# Autodesk Inventor assembly: Calorímetro
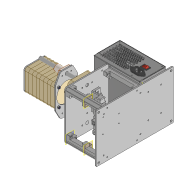
[picture p0: Inventor's stored thumbnail of the model, 180x180]
Saved by Autodesk Inventor 2020 (Build 240168000, 168)
## iProperties
Created: 2022-07-16
Part Number: Calorímetro
Document SubType Name: Assembly
Designer: gabri
Author: gabri
## Documents named in this file (11)
- C:\Users\gabri\OneDrive\Área de Trabalho\Calorimetro 2022\Inventor\Calorímetro.iam
- C:\Users\gabri\OneDrive\Área de Trabalho\Calorimetro 2022\Inventor\Fonte\ATX Power Supply v1.iam
- C:\Users\gabri\OneDrive\Área de Trabalho\Calorimetro 2022\Inventor\Base.ipt
- C:\Users\gabri\OneDrive\Área de Trabalho\Calorimetro 2022\Inventor\parte_superior.iam
- C:\Users\gabri\OneDrive\Área de Trabalho\Calorimetro 2022\Inventor\Montagem_suporte_termopar.iam
- C:\Users\gabri\OneDrive\Área de Trabalho\Calorimetro 2022\Inventor\Peça4.ipt
- C:\Users\gabri\OneDrive\Área de Trabalho\Calorimetro 2022\Inventor\suporte-fonte.ipt
- C:\Users\gabri\OneDrive\Área de Trabalho\Calorimetro 2022\Inventor\suporte_fechamento.ipt
- C:\Users\gabri\OneDrive\Área de Trabalho\Calorimetro 2022\Inventor\suporte_fechamento2.ipt
- C:\Users\gabri\OneDrive\Área de Trabalho\Calorimetro 2022\Inventor\fechamentocima.ipt
- C:\Users\gabri\OneDrive\Área de Trabalho\Calorimetro 2022\Inventor\Mega.ipt
## Components (12 placed, 10 different names)
1. ATX Power Supply v1:1 [sub-assembly] — Coincidência:1, Alinhamento:1, Coincidência:2, Coincidência:5, Coincidência:6, Alinhamento:4, Alinhamento:5, Alinhamento:6, Alinhamento:7
2. Base:1 — Coincidência:7, Alinhamento:6, Alinhamento:7, Coincidência:8, Coincidência:9, Alinhamento:8, Alinhamento:9, Alinhamento:10, Alinhamento:12, Coincidência:10, Coincidência:12, Coincidência:16, Alinhamento:19, Alinhamento:20
3. parte_superior:1 [sub-assembly] — Coincidência:4, Alinhamento:2, Coincidência:13, Alinhamento:17, Alinhamento:18, Coincidência:14
4. Montagem_suporte_termopar:1 [sub-assembly] — Coincidência:4, Coincidência:14, Coincidência:15, Ângulo:1
5. Peça4:1 — Alinhamento:2
6. suporte-fonte:1 — Coincidência:5, Coincidência:6, Coincidência:7, Alinhamento:4, Alinhamento:5, Coincidência:11
7. suporte_fechamento:1 — Coincidência:8, Alinhamento:8, Alinhamento:11, Alinhamento:15
8. suporte_fechamento:2 — Coincidência:9, Alinhamento:9, Alinhamento:10, Alinhamento:11, Alinhamento:13, Alinhamento:16
9. suporte_fechamento2:2 — Alinhamento:12, Coincidência:10, Coincidência:11, Alinhamento:14
10. suporte_fechamento2:3 — Coincidência:12, Alinhamento:13, Alinhamento:14
11. fechamentocima:1 — Alinhamento:15, Alinhamento:16, Coincidência:13, Alinhamento:17, Alinhamento:18, Coincidência:15, Ângulo:1
12. Mega:1 — Coincidência:16, Alinhamento:19, Alinhamento:20
## Relationships (35: Flush 19, Mate 15, Angle 1)
- Coincidência:1 [Mate] (-71 mm): ATX Power Supply v1:1
- Alinhamento:1 [Flush]: ATX Power Supply v1:1
- Coincidência:2 [Mate]: ATX Power Supply v1:1
- Coincidência:4 [Mate]: parte_superior:1 ↔ Montagem_suporte_termopar:1
- Alinhamento:2 [Flush]: parte_superior:1 ↔ Peça4:1
- Coincidência:5 [Mate]: ATX Power Supply v1:1 ↔ suporte-fonte:1
- Coincidência:6 [Mate]: ATX Power Supply v1:1 ↔ suporte-fonte:1
- Coincidência:7 [Mate]: Base:1 ↔ suporte-fonte:1
- Alinhamento:4 [Flush]: ATX Power Supply v1:1 ↔ suporte-fonte:1
- Alinhamento:5 [Flush] (-8 mm): ATX Power Supply v1:1 ↔ suporte-fonte:1
- Alinhamento:6 [Flush] (-13 mm): ATX Power Supply v1:1 ↔ Base:1
- Alinhamento:7 [Flush]: ATX Power Supply v1:1 ↔ Base:1
- Coincidência:8 [Mate]: Base:1 ↔ suporte_fechamento:1
- Coincidência:9 [Mate]: Base:1 ↔ suporte_fechamento:2
- Alinhamento:8 [Flush]: Base:1 ↔ suporte_fechamento:1
- Alinhamento:9 [Flush]: Base:1 ↔ suporte_fechamento:2
- Alinhamento:10 [Flush] (15 mm): Base:1 ↔ suporte_fechamento:2
- Alinhamento:11 [Flush]: suporte_fechamento:1 ↔ suporte_fechamento:2
- Alinhamento:12 [Flush]: Base:1 ↔ suporte_fechamento2:2
- Coincidência:10 [Mate]: Base:1 ↔ suporte_fechamento2:2
- Coincidência:11 [Mate]: suporte-fonte:1 ↔ suporte_fechamento2:2
- Coincidência:12 [Mate]: Base:1 ↔ suporte_fechamento2:3
- Alinhamento:13 [Flush]: suporte_fechamento:2 ↔ suporte_fechamento2:3
- Alinhamento:14 [Flush]: suporte_fechamento2:2 ↔ suporte_fechamento2:3
- Alinhamento:15 [Flush]: suporte_fechamento:1 ↔ fechamentocima:1
- Alinhamento:16 [Flush]: suporte_fechamento:2 ↔ fechamentocima:1
- Coincidência:13 [Mate]: parte_superior:1 ↔ fechamentocima:1
- Alinhamento:17 [Flush] (33.5 mm): parte_superior:1 ↔ fechamentocima:1
- Alinhamento:18 [Flush] (12.82 mm): parte_superior:1 ↔ fechamentocima:1
- Coincidência:14 [Mate]: parte_superior:1 ↔ Montagem_suporte_termopar:1
- Coincidência:15 [Mate]: Montagem_suporte_termopar:1 ↔ fechamentocima:1
- Ângulo:1 [Angle] (0 deg): Montagem_suporte_termopar:1 ↔ fechamentocima:1
- Coincidência:16 [Mate]: Base:1 ↔ Mega:1
- Alinhamento:19 [Flush] (3 mm): Base:1 ↔ Mega:1
- Alinhamento:20 [Flush] (26 mm): Base:1 ↔ Mega:1
